# Autodesk Inventor assembly: 採果車初版
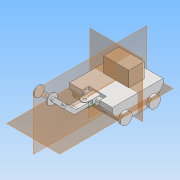
[picture p0: Inventor's stored thumbnail of the model, 180x180]
Saved by Autodesk Inventor 2021 (Build 250183000, 183)
## iProperties
Created: 2025-12-12
Part Number: 採果車初版
Document SubType Name: Assembly
Designer: User
Author: User
## Documents named in this file (12)
- C:\Users\User\Documents\Inventor\Projects\採果車\採果車初版.iam
- C:\Users\User\Documents\Inventor\Projects\採果車\車身.ipt
- C:\Users\User\Documents\Inventor\Projects\採果車\車體上做.ipt
- C:\Users\User\Documents\Inventor\Projects\採果車\萬象塊.ipt
- C:\Users\User\Documents\Inventor\Projects\採果車\滾珠軸承(標準).ipt
- C:\Users\User\Documents\Inventor\Projects\採果車\車輪.ipt
- C:\Users\User\Documents\Inventor\Projects\採果車\主吊臂.ipt
- C:\Users\User\Documents\Inventor\Projects\採果車\震動臂.ipt
- C:\Users\User\Documents\Inventor\Projects\採果車\夾緊支撐感.ipt
- C:\Users\User\Documents\Inventor\Projects\採果車\夾緊船動感.ipt
- C:\Users\User\Documents\Inventor\Projects\採果車\偏心倫.ipt
- C:\Users\User\Documents\Inventor\Projects\採果車\特規趁套.ipt
## Components (19 placed, 11 different names)
1. 車身:1 — 貼合:1, 角度:1, 貼合:2, 齊平:4, 齊平:5, 貼合:3, 齊平:6, 貼合:4, 齊平:7, 貼合:5
2. 車體上做:1 — 齊平:1, 齊平:2
3. 萬象塊:1 — 齊平:3, 貼合:1, 角度:1, 角度:2, 插入:10
4. 滾珠軸承(標準):1 — 貼合:2, 齊平:4, 插入:1
5. 滾珠軸承(標準):2 — 齊平:5, 貼合:3, 插入:2
6. 滾珠軸承(標準):3 — 齊平:6, 貼合:4, 插入:4
7. 滾珠軸承(標準):4 — 齊平:7, 貼合:5, 插入:3
8. 車輪:1 — 插入:1
9. 車輪:2 — 插入:2
10. 車輪:3 — 插入:3
11. 車輪:4 — 插入:4
12. 主吊臂:1 — 角度:2, 貼合:6, 貼合:7, 貼合:8, 貼合:9, 貼合:10, 插入:11
13. 震動臂:1 — 貼合:6, 貼合:7, 插入:6, 插入:8, 插入:9
14. 震動臂:2 — 貼合:8, 貼合:9, 插入:7
15. 夾緊支撐感:1 — 插入:6, 插入:7
16. 夾緊船動感:1 — 插入:8
17. 夾緊船動感:2 — 插入:9
18. 偏心倫:1 — 貼合:10
19. 特規趁套:1 — 插入:10, 插入:11
## Relationships (29: Mate 10, Insert 10, Flush 7, Angle 2)
- 齊平:1 [Flush]: 車體上做:1
- 齊平:2 [Flush]: 車體上做:1
- 齊平:3 [Flush]: 萬象塊:1
- 貼合:1 [Mate]: 車身:1 ↔ 萬象塊:1
- 角度:1 [Angle] (0 deg): 車身:1 ↔ 萬象塊:1
- 貼合:2 [Mate]: 車身:1 ↔ 滾珠軸承(標準):1
- 齊平:4 [Flush]: 車身:1 ↔ 滾珠軸承(標準):1
- 齊平:5 [Flush]: 車身:1 ↔ 滾珠軸承(標準):2
- 貼合:3 [Mate]: 車身:1 ↔ 滾珠軸承(標準):2
- 齊平:6 [Flush]: 車身:1 ↔ 滾珠軸承(標準):3
- 貼合:4 [Mate]: 車身:1 ↔ 滾珠軸承(標準):3
- 齊平:7 [Flush]: 車身:1 ↔ 滾珠軸承(標準):4
- 貼合:5 [Mate]: 車身:1 ↔ 滾珠軸承(標準):4
- 插入:1 [Insert]: 滾珠軸承(標準):1 ↔ 車輪:1
- 插入:2 [Insert]: 滾珠軸承(標準):2 ↔ 車輪:2
- 插入:3 [Insert]: 滾珠軸承(標準):4 ↔ 車輪:3
- 插入:4 [Insert]: 滾珠軸承(標準):3 ↔ 車輪:4
- 角度:2 [Angle] (0 deg): 萬象塊:1 ↔ 主吊臂:1
- 貼合:6 [Mate]: 主吊臂:1 ↔ 震動臂:1
- 貼合:7 [Mate]: 主吊臂:1 ↔ 震動臂:1
- 貼合:8 [Mate]: 主吊臂:1 ↔ 震動臂:2
- 貼合:9 [Mate]: 主吊臂:1 ↔ 震動臂:2
- 插入:6 [Insert]: 震動臂:1 ↔ 夾緊支撐感:1
- 插入:7 [Insert]: 震動臂:2 ↔ 夾緊支撐感:1
- 插入:8 [Insert]: 震動臂:1 ↔ 夾緊船動感:1
- 插入:9 [Insert]: 震動臂:1 ↔ 夾緊船動感:2
- 貼合:10 [Mate]: 主吊臂:1 ↔ 偏心倫:1
- 插入:10 [Insert]: 萬象塊:1 ↔ 特規趁套:1
- 插入:11 [Insert]: 主吊臂:1 ↔ 特規趁套:1
